# Autodesk Inventor assembly: 100-10-FRAME-ROCKER-SCREW-01
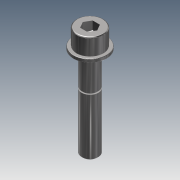
[picture p0: Inventor's stored thumbnail of the model, 180x180]
Saved by Autodesk Inventor 2018.2 (Build 222227000, 227)
## iProperties
Manager: feesmrt
Company: FRANCOR
Part Number: 100-10-FRAME-ROCKER-SCREW-01
Project: Rescue Robot
Cost Center: -
Material: Generisch
Document SubType Name: Assembly
Designer: feesmrt
Engineer: feesmrt
Authority: feesmrt
Description: Rockerbearing Screw and Washer
Stock Number: 100-10-FRAME-ROCKER-SCREW-01
Subject: Rescue Robot
Author: feesmrt
Revision Number: 1
Title: Rockerbearing Screw and Washer
## Documents named in this file (3)
- D:\Programmierung\FRANC0R\CAD\02-Rocker-Bogie-Robot\100-CHASSIS\10-FRAME\100-10-FRAME-ROCKER-SCREW-01.iam
- D:\Programmierung\FRANC0R\CAD\02-Rocker-Bogie-Robot\900-COMPONENTS\900-80-WASHERS\900-80-WASHERS-ISO7091-8.ipt
- D:\Programmierung\FRANC0R\CAD\02-Rocker-Bogie-Robot\900-COMPONENTS\900-40-SCREWS\900-40-SCREWS-ISO4762_M8x45.ipt
## Components (2 placed, 2 different names)
1. 900-40-SCREWS-ISO4762_M8x45:1 — Passend:1, Passend:2
2. 900-80-WASHERS-ISO7091-8:1 — Passend:1, Passend:2
## Relationships (2: Mate 2)
- Passend:1 [Mate]: 900-40-SCREWS-ISO4762_M8x45:1 ↔ 900-80-WASHERS-ISO7091-8:1
- Passend:2 [Mate]: 900-40-SCREWS-ISO4762_M8x45:1 ↔ 900-80-WASHERS-ISO7091-8:1
